# Autodesk Inventor assembly: licht_50
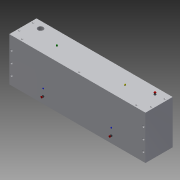
[picture p0: Inventor's stored thumbnail of the model, 180x180]
Saved by Autodesk Inventor 2015 (Build 190159000, 159)
## iProperties
Created: 2018-01-11
Part Number: licht_50
Document SubType Name: Assembly
Designer: schueler
Author: schueler
## Documents named in this file (8)
- C:\workspace\robosax\licht\Teamprobe\licht_50.iam
- C:\workspace\robosax\licht\Teamprobe\licht_50_front.ipt
- C:\workspace\robosax\licht\Teamprobe\licht_50_top.ipt
- C:\workspace\robosax\licht\Teamprobe\licht_side_simple.ipt
- C:\workspace\robosax\licht_temp\licht_taster.ipt
- C:\workspace\robosax\licht_temp\licht_led_blau.ipt
- C:\workspace\robosax\licht_temp\licht_led_gelb.ipt
- C:\workspace\robosax\licht_temp\licht_led_gruen.ipt
## Components (11 placed, 7 different names)
1. licht_50_front:1 — Fluchtend:1, Passend:1, Fluchtend:2, Passend:2, Fluchtend:3, Passend:4, Passend:5, Passend:6, Passend:7, Fluchtend:4, Einfügen:1, Einfügen:2, Einfügen:4, Einfügen:5
2. licht_50_top:1 — Fluchtend:1, Passend:1, Fluchtend:2, Passend:3, Passend:8, Einfügen:3, Einfügen:6, Einfügen:7
3. licht_side_simple:1 — Passend:7, Passend:8, Fluchtend:4
4. licht_side_simple:2 — Passend:2, Passend:3, Fluchtend:3
5. licht_taster:1 — Einfügen:1
6. licht_taster:2 — Einfügen:2
7. licht_taster:3 — Einfügen:3
8. licht_led_blau:1 — Einfügen:4
9. licht_led_blau:2 — Einfügen:5
10. licht_led_gelb:1 — Einfügen:7
11. licht_led_gruen:1 — Einfügen:6
## Relationships (19: Mate 8, Insert 7, Flush 4)
- Fluchtend:1 [Flush]: licht_50_front:1 ↔ licht_50_top:1
- Passend:1 [Mate]: licht_50_front:1 ↔ licht_50_top:1
- Fluchtend:2 [Flush]: licht_50_front:1 ↔ licht_50_top:1
- Passend:2 [Mate]: licht_50_front:1 ↔ licht_side_simple:2
- Passend:3 [Mate]: licht_50_top:1 ↔ licht_side_simple:2
- Fluchtend:3 [Flush]: licht_50_front:1 ↔ licht_side_simple:2
- Passend:4 [Mate]: licht_50_front:1
- Passend:5 [Mate]: licht_50_front:1
- Passend:6 [Mate]: licht_50_front:1
- Passend:7 [Mate]: licht_50_front:1 ↔ licht_side_simple:1
- Passend:8 [Mate]: licht_50_top:1 ↔ licht_side_simple:1
- Fluchtend:4 [Flush]: licht_50_front:1 ↔ licht_side_simple:1
- Einfügen:1 [Insert] (-14 mm): licht_50_front:1 ↔ licht_taster:1
- Einfügen:2 [Insert] (-6 mm): licht_50_front:1 ↔ licht_taster:2
- Einfügen:3 [Insert] (-8 mm): licht_50_top:1 ↔ licht_taster:3
- Einfügen:4 [Insert]: licht_50_front:1 ↔ licht_led_blau:1
- Einfügen:5 [Insert]: licht_50_front:1 ↔ licht_led_blau:2
- Einfügen:6 [Insert] (2 mm): licht_50_top:1 ↔ licht_led_gruen:1
- Einfügen:7 [Insert] (2 mm): licht_50_top:1 ↔ licht_led_gelb:1
